# Autodesk Inventor assembly: Fixture Assembly
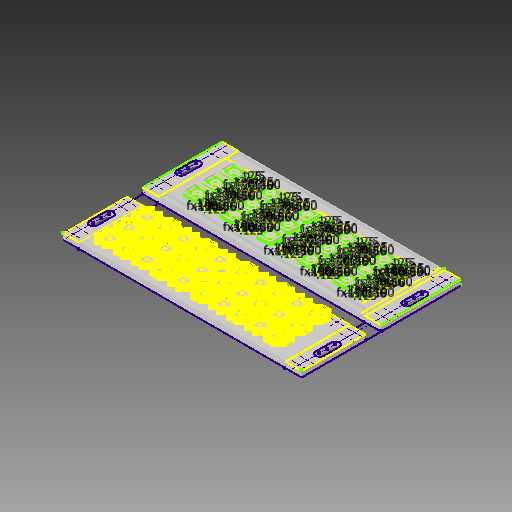
[picture p0: Inventor's stored thumbnail of the model, 512x512]
Saved by Autodesk Inventor 2018 (Build 220112000, 112)
## iProperties
Created: 2016-04-08
Part Number: Fixture Assembly
Document SubType Name: Assembly
Designer: Sam Clay
Author: Sam Clay
## Documents named in this file (6)
- Z:\enclosure\inventor\Fixture Assembly.iam
- Z:\enclosure\inventor\Fixture Base.ipt
- Z:\enclosure\inventor\Case Top.ipt
- Z:\enclosure\inventor\Case Bottom.ipt
- Z:\enclosure\inventor\Case Top Fixture.ipt
- Z:\enclosure\inventor\Case Bottom Fixture.ipt
## Components (61 placed, 5 different names)
1. Fixture Base:1 — Mate:12, Mate:13, Mate:15, Mate:16, Mate:18, Mate:26, Mate:27, Mate:28, Mate:30
2. Case Bottom:1 — Mate top pocket shell, Mate side pocket shell
3. Case Bottom:2
4. Case Bottom:3
5. Case Bottom:4
6. Case Bottom:5
7. Case Bottom:6
8. Case Top:2 — Mate side pocket shell, Mate top pocket shell, Mate:12, Mate:15, Mate:30, Mate:17
9. Case Top:3
10. Case Top:4
11. Case Top:5
12. Case Top:6
13. Case Top:7
14. Case Top:8
15. Case Top:9
16. Case Top:10
17. Case Top Fixture:1 — Mate:26, Mate:27, Mate:28, Mate:31, Mate:32, Mate:29
18. Case Top Fixture:2
19. Case Top Fixture:3
20. Case Top Fixture:4
21. Case Top Fixture:5
22. Case Top Fixture:6
23. Case Top Fixture:7 — Mate:23
24. Case Top Fixture:8
25. Case Top Fixture:9
26. Case Bottom:7 — Mate top pocket shell 2, Mate:13, Mate:16, Mate:17, Mate:19
27. Case Bottom:8
28. Case Bottom:9
29. Case Bottom:10
30. Case Bottom:11
31. Case Bottom:12
32. Case Bottom:13
33. Case Bottom:14
34. Case Bottom:15
35. Case Top:11 — Mate top pocket shell 2, Mate:18, Mate:19
36. Case Top:12
37. Case Top:13
38. Case Top:14
39. Case Top:15
40. Case Top:16
41. Case Bottom Fixture:7 — Mate:21, Mate:22, Mate:23, Mate:29
42. Case Bottom Fixture:8
43. Case Bottom Fixture:9
44. Case Bottom Fixture:10
45. Case Bottom Fixture:11
46. Case Bottom Fixture:12
47. Case Bottom Fixture:13
48. Case Bottom Fixture:14
49. Case Bottom Fixture:15
50. Case Top Fixture:10 — Mate:21, Mate:22
51. Case Top Fixture:11
52. Case Top Fixture:12
53. Case Top Fixture:13
54. Case Top Fixture:14
55. Case Top Fixture:15
56. Case Bottom Fixture:16 — Mate:31, Mate:32
57. Case Bottom Fixture:17
58. Case Bottom Fixture:18
59. Case Bottom Fixture:19
60. Case Bottom Fixture:20
61. Case Bottom Fixture:21
## Component patterns: (6 elements, first: Case Bottom:1), (9 elements, first: Case Top:2), (9 elements, first: Case Top Fixture:1), (9 elements, first: Case Bottom:7), (6 elements, first: Case Top:11), (9 elements, first: Case Bottom Fixture:7), (6 elements, first: Case Top Fixture:10), (6 elements, first: Case Bottom Fixture:16)
## Relationships (20: Mate 20)
- Mate top pocket shell: Case Bottom:1 ↔ Case Top:2
- Mate top pocket shell 2: Case Bottom:7 ↔ Case Top:11
- Mate side pocket shell (6.604 mm): Case Bottom:1 ↔ Case Top:2
- Mate:12: Fixture Base:1 ↔ Case Top:2
- Mate:13: Fixture Base:1 ↔ Case Bottom:7
- Mate:15 (3.175 mm): Fixture Base:1 ↔ Case Top:2
- Mate:16 (1.27 mm): Fixture Base:1 ↔ Case Bottom:7
- Mate:17 (304.8 mm): Case Top:2 ↔ Case Bottom:7
- Mate:19 (6.604 mm): Case Bottom:7 ↔ Case Top:11
- Mate:18: Fixture Base:1 ↔ Case Top:11
- Mate:21: Case Bottom Fixture:7 ↔ Case Top Fixture:10
- Mate:22 (6.604 mm): Case Bottom Fixture:7 ↔ Case Top Fixture:10
- Mate:23: Case Top Fixture:7 ↔ Case Bottom Fixture:7
- Mate:26 (16.51 mm): Fixture Base:1 ↔ Case Top Fixture:1
- Mate:27 (24.13 mm): Fixture Base:1 ↔ Case Top Fixture:1
- Mate:28 (41.91 mm): Fixture Base:1 ↔ Case Top Fixture:1
- Mate:29 (304.8 mm): Case Top Fixture:1 ↔ Case Bottom Fixture:7
- Mate:30 (1.27 mm): Fixture Base:1 ↔ Case Top:2
- Mate:31: Case Top Fixture:1 ↔ Case Bottom Fixture:16
- Mate:32 (6.604 mm): Case Top Fixture:1 ↔ Case Bottom Fixture:16
